# Autodesk Inventor assembly: MovingPlate
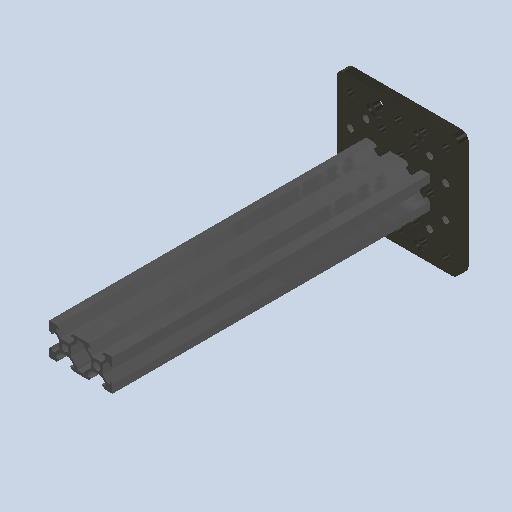
[picture p0: Inventor's stored thumbnail of the model, 512x512]
Saved by Autodesk Inventor 2024.2 (Build 282272000, 272)
## iProperties
Created: 2024-08-27
Part Number: MovingPlate
Document SubType Name: Assembly
Designer: Admin
Author: Admin
## Documents named in this file (5)
- C:\Users\Admin\Documents\GitHub\ManipuladorCartesiano\DiseñoMecánico\Assemblies\MovingPlate.iam
- C:\Users\Admin\Documents\GitHub\ManipuladorCartesiano\DiseñoMecánico\Axis\AxisZ\MovingPlate\AntiBacklashBlock.ipt
- C:\Users\Admin\Documents\GitHub\ManipuladorCartesiano\DiseñoMecánico\Axis\AxisZ\MovingPlate\AluminiumSpacer3mm.ipt
- C:\Users\Admin\Documents\GitHub\ManipuladorCartesiano\DiseñoMecánico\Axis\AxisZ\MovingPlate\C-BeamPlate.ipt
- C:\Users\Admin\Documents\GitHub\ManipuladorCartesiano\DiseñoMecánico\Axis\AxisZ\MovingPlate\AP-ZClaw.ipt
## Components (5 placed, 4 different names)
1. AntiBacklashBlock:1 — Mate:1, Mate:2, Mate:3, Mate:4
2. AluminiumSpacer3mm:1 — Mate:3, Mate:4, Mate:5, Mate:7
3. AluminiumSpacer3mm:2 — Mate:1, Mate:2, Mate:6
4. C-BeamPlate:1 — Mate:5, Mate:6, Mate:7, Mate:9, Mate:10, Mate:11
5. AP-ZClaw:1 — Mate:9, Mate:10, Mate:11
## Relationships (10: Mate 10)
- Mate:1: AntiBacklashBlock:1 ↔ AluminiumSpacer3mm:2
- Mate:2: AntiBacklashBlock:1 ↔ AluminiumSpacer3mm:2
- Mate:3: AntiBacklashBlock:1 ↔ AluminiumSpacer3mm:1
- Mate:4: AntiBacklashBlock:1 ↔ AluminiumSpacer3mm:1
- Mate:5: AluminiumSpacer3mm:1 ↔ C-BeamPlate:1
- Mate:6: AluminiumSpacer3mm:2 ↔ C-BeamPlate:1
- Mate:7: AluminiumSpacer3mm:1 ↔ C-BeamPlate:1
- Mate:9: C-BeamPlate:1 ↔ AP-ZClaw:1
- Mate:10: C-BeamPlate:1 ↔ AP-ZClaw:1
- Mate:11: C-BeamPlate:1 ↔ AP-ZClaw:1
